# Autodesk Inventor assembly: MotorRail
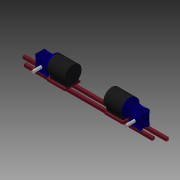
[picture p0: Inventor's stored thumbnail of the model, 180x180]
Saved by Autodesk Inventor 2015 SP1 (Build 190203100, 203)
## iProperties
Created: 2016-03-21
Part Number: MotorRail
Document SubType Name: Assembly
Designer: Mac
Author: Mac
## Documents named in this file (8)
- C:\Users\jonesdm\Desktop\MotionBase\CAD\MotionBaseCAD\MotorRail.iam
- C:\Users\jonesdm\Desktop\MotionBase\CAD\MotionBaseCAD\1inSquareSupport2.ipt
- C:\Users\jonesdm\Desktop\MotionBase\CAD\MotionBaseCAD\1inSquareSupportOut.ipt
- C:\Users\jonesdm\Desktop\MotionBase\CAD\MotionBaseCAD\Motor4.ipt
- C:\Users\jonesdm\Desktop\MotionBase\CAD\MotionBaseCAD\Imported Components\WGA-50M-080-H1\WGA-50M-080-H1.ipt
- C:\Users\jonesdm\Desktop\MotionBase\CAD\MotionBaseCAD\GearShaft.ipt
- C:\Users\jonesdm\Desktop\MotionBase\CAD\MotionBaseCAD\MotionBaseGeneric.iam
- C:\Users\jonesdm\Desktop\MotionBase\CAD\MotionBaseCAD\Motor Shim.ipt
## Components (10 placed, 6 different names)
1. 1inSquareSupport2:1 — Mate:7, Mate:16, Flush:9, Mate:17, Symmetry:2, Mate:19, Mate:20, Mate:21
2. 1inSquareSupportOut:1 — Mate:6, Flush:8, Flush:10, Symmetry:2
3. Motor4:1 — Mate:1, Mate:2, Angle:1, Mate:15, Symmetry:1, Flush:13
4. WGA-50M-080-H1:1 — Mate:1, Mate:2, Angle:1, Mate:3, Mate:4, Flush:1, Mate:6, Mate:7, Flush:6, Flush:7, Flush:8, Mate:16, Flush:9
5. GearShaft:1 — Mate:3, Mate:4, Flush:1
6. Motor4:2 — Mate:15, Symmetry:1, Flush:12
7. WGA-50M-080-H1:2 — Mate:13, Flush:5, Mate:14, Flush:6, Flush:7
8. GearShaft:2 — Mate:13, Flush:5, Mate:14
9. Motor Shim:1 — Mate:21, Mate:22, Flush:13
10. Motor Shim:2 — Mate:20, Mate:23, Flush:12
## Relationships (33: Mate 19, Flush 10, Angle 2, Symmetry 2)
- Mate:1: Motor4:1 ↔ WGA-50M-080-H1:1
- Mate:2: Motor4:1 ↔ WGA-50M-080-H1:1
- Angle:1 (0 deg): Motor4:1 ↔ WGA-50M-080-H1:1
- Mate:3: WGA-50M-080-H1:1 ↔ GearShaft:1
- Mate:4: WGA-50M-080-H1:1 ↔ GearShaft:1
- Flush:1 (50.8 mm): WGA-50M-080-H1:1 ↔ GearShaft:1
- Mate:6: 1inSquareSupportOut:1 ↔ WGA-50M-080-H1:1
- Mate:7: 1inSquareSupport2:1 ↔ WGA-50M-080-H1:1
- [Mate]: Motor4:2 ↔ WGA-50M-080-H1:2
- [Mate]: Motor4:2 ↔ WGA-50M-080-H1:2
- [Angle] (0 deg): Motor4:2 ↔ WGA-50M-080-H1:2
- Mate:13: WGA-50M-080-H1:2 ↔ GearShaft:2
- Flush:5 (50.8 mm): WGA-50M-080-H1:2 ↔ GearShaft:2
- Mate:14: WGA-50M-080-H1:2 ↔ GearShaft:2
- Mate:15 (381 mm): Motor4:1 ↔ Motor4:2
- Flush:6: WGA-50M-080-H1:1 ↔ WGA-50M-080-H1:2
- Flush:7: WGA-50M-080-H1:1 ↔ WGA-50M-080-H1:2
- Flush:8 (-1.8479 mm): 1inSquareSupportOut:1 ↔ WGA-50M-080-H1:1
- Mate:16: 1inSquareSupport2:1 ↔ WGA-50M-080-H1:1
- Flush:9 (-1.8479 mm): 1inSquareSupport2:1 ↔ WGA-50M-080-H1:1
- Symmetry:1: Motor4:1 ↔ Motor4:2
- Mate:17: 1inSquareSupport2:1
- Flush:10: 1inSquareSupportOut:1
- Flush:11
- Symmetry:2: 1inSquareSupport2:1 ↔ 1inSquareSupportOut:1
- Mate:18
- Mate:19: 1inSquareSupport2:1
- Mate:20: 1inSquareSupport2:1 ↔ Motor Shim:2
- Mate:21: 1inSquareSupport2:1 ↔ Motor Shim:1
- Mate:22: Motor Shim:1
- Mate:23: Motor Shim:2
- Flush:12: Motor4:2 ↔ Motor Shim:2
- Flush:13: Motor4:1 ↔ Motor Shim:1
## Named parameters: d15_d0 = 0 mm, d16_d1 = 0 mm, d17_d2 = 0 deg, math = 3.6957 mm
